# Autodesk Inventor assembly: Вентилятор 92x92x25
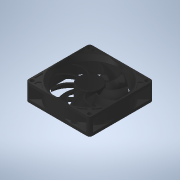
[picture p0: Inventor's stored thumbnail of the model, 180x180]
Saved by Autodesk Inventor 2021.2 (Build 252289000, 289)
## iProperties
Created: 2021-09-06
Part Number: Вентилятор 92x92x25
Document SubType Name: Assembly
Designer: asus
Mass: 78.6028 g
Surface Area: 463.439 cm^2
Volume: 74.1536 cm^3
Density: 1.06 g/cm^3
Author: asus
## Documents named in this file (3)
- C:\Users\asus\Desktop\inventor\PC_components\Вентилятор 90x90x25\Вентилятор 92x92x25.iam
- C:\Users\asus\Desktop\inventor\PC_components\Вентилятор 90x90x25\Вентилятор_винт 92x92x25.ipt
- C:\Users\asus\Desktop\inventor\PC_components\Вентилятор 90x90x25\Вентилятор_основа 92x92x25.ipt
## Components (2 placed, 2 different names)
1. Вентилятор_винт 92x92x25:1 — С поворотом:1
2. Вентилятор_основа 92x92x25:1 — С поворотом:1
## Relationships (1: RevoluteJoint 1)
- С поворотом:1 [RevoluteJoint]: Вентилятор_винт 92x92x25:1 ↔ Вентилятор_основа 92x92x25:1
